(part 1 of 3)
# Autodesk Inventor assembly: CNC-FullAssembly
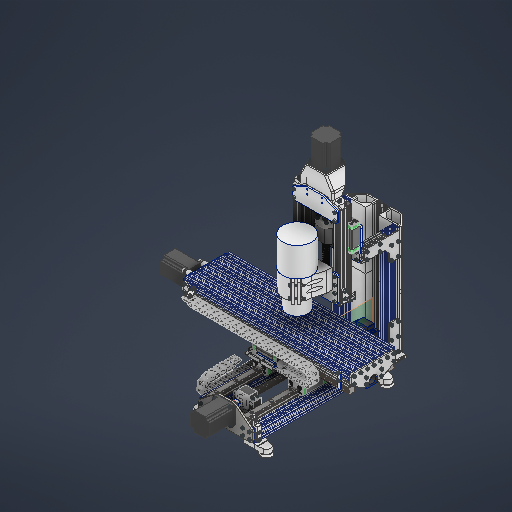
[picture p0: Inventor's stored thumbnail of the model, 512x512]
Saved by Autodesk Inventor 2026.2 (Build 302298000, 298)
## iProperties
Created: 2026-06-14
Part Number: CNC-FullAssembly
Document SubType Name: Assembly
Designer: Kenji
Mass: 17887.4 g
Surface Area: 25590.9 cm^2
Volume: 4676.24 cm^3
Author: Kenji
## Documents named in this file (79)
- C:\Users\Kenji\Documents\GitHub\DiyCNC-\CNC-FullAssembly.iam
- C:\Users\Kenji\Documents\GitHub\DiyCNC-\COTS-Parts\40x40x500mm-Extrusion.ipt
- C:\Users\Kenji\Documents\GitHub\DiyCNC-\COTS-Parts\SFU1605-BallScrewNut.iam
- C:\Users\Kenji\Documents\GitHub\DiyCNC-\COTS-Parts\DSG16H-BallScrewFixtureBlock.ipt
- C:\Users\Kenji\Documents\GitHub\DiyCNC-\COTS-Parts\SFU1605-BallScrew500mm.ipt
- C:\Users\Kenji\Documents\GitHub\DiyCNC-\COTS-Parts\BK12-BallScrewStabilizer.iam
- C:\Users\Kenji\Documents\GitHub\DiyCNC-\COTS-Parts\HGR20R-LinearRail500mm.ipt
- C:\Users\Kenji\Documents\GitHub\DiyCNC-\COTS-Parts\HGH20-LinearRailCarriage.iam
- C:\Users\Kenji\Documents\GitHub\DiyCNC-\COTS-Parts\91274A131_M5x20mm.ipt
- C:\Users\Kenji\Documents\GitHub\DiyCNC-\COTS-Parts\91290A231-M5x15mm.ipt
- C:\Users\Kenji\Documents\GitHub\DiyCNC-\COTS-Parts\Nema23-StepperMotor.ipt
- C:\Users\Kenji\Documents\GitHub\DiyCNC-\COTS-Parts\MH2025-6.35x10mmCoupler.iam
- C:\Users\Kenji\Documents\GitHub\DiyCNC-\COTS-Parts\BF12-BallScrewStabilizer2.ipt
- C:\Users\Kenji\Documents\GitHub\DiyCNC-\CNC-000-StructureGusset1.ipt
- C:\Users\Kenji\Documents\GitHub\DiyCNC-\COTS-Parts\20x40x500mm-Extrusion.ipt
- C:\Users\Kenji\Documents\GitHub\DiyCNC-\CNC-001-StructureGusset2.ipt
- C:\Users\Kenji\Documents\GitHub\DiyCNC-\CNC-002-ShimStructureGusset2.ipt
- C:\Users\Kenji\Documents\GitHub\DiyCNC-\COTS-Parts\90576A104-M5-NylockNut.ipt
- C:\Users\Kenji\Documents\GitHub\DiyCNC-\COTS-Parts\91292A195-M5x45mm.ipt
- C:\Users\Kenji\Documents\GitHub\DiyCNC-\CNC-003-StructureGusset3.ipt
- C:\Users\Kenji\Documents\GitHub\DiyCNC-\CNC-004-Nema23Shim.ipt
- C:\Users\Kenji\Documents\GitHub\DiyCNC-\COTS-Parts\91274A125-M5x8mm.ipt
- C:\Users\Kenji\Documents\GitHub\DiyCNC-\CNC-005-XAxisMount1.ipt
- C:\Users\Kenji\Documents\GitHub\DiyCNC-\COTS-Parts\91263A832-M5x10mm-Countersink.ipt
- C:\Users\Kenji\Documents\GitHub\DiyCNC-\CNC-006-XAxisMount2.ipt
- C:\Users\Kenji\Documents\GitHub\DiyCNC-\COTS-Parts\92095A495-M8-18mm-ButtonHead.ipt
- C:\Users\Kenji\Documents\GitHub\DiyCNC-\COTS-Parts\94645A210-M8-NylockNut.ipt
- C:\Users\Kenji\Documents\GitHub\DiyCNC-\COTS-Parts\20x40x500mm-Extrusion2.ipt
- C:\Users\Kenji\Documents\GitHub\DiyCNC-\COTS-Parts\20x20x500mm_Extrusion.ipt
- C:\Users\Kenji\Documents\GitHub\DiyCNC-\CNC-007-XAxisBallScrewMount.ipt
- C:\Users\Kenji\Documents\GitHub\DiyCNC-\CNC-008-XAxisNema23Mount.ipt
- C:\Users\Kenji\Documents\GitHub\DiyCNC-\CNC-009-XAxisNema23Spacer.ipt
- C:\Users\Kenji\Documents\GitHub\DiyCNC-\COTS-Parts\91290A198-M5-50mm.ipt
- C:\Users\Kenji\Documents\GitHub\DiyCNC-\COTS-Parts\3103-0001-0002-GobildaLimitSwitch.ipt
- C:\Users\Kenji\Documents\GitHub\DiyCNC-\CNC-010-XAxisLimitSwitchMount.ipt
- C:\Users\Kenji\Documents\GitHub\DiyCNC-\CNC-011-XAxisHardStop.ipt
- C:\Users\Kenji\Documents\GitHub\DiyCNC-\COTS-Parts\HGR20R-LinearRail300mm.ipt
- C:\Users\Kenji\Documents\GitHub\DiyCNC-\COTS-Parts\SFU1605-BallScrew400mm.ipt
- C:\Users\Kenji\Documents\GitHub\DiyCNC-\COTS-Parts\RouterSpindle-65mm.ipt
- C:\Users\Kenji\Documents\GitHub\DiyCNC-\COTS-Parts\90128A046-#2-.375in.ipt
- C:\Users\Kenji\Documents\GitHub\DiyCNC-\COTS-Parts\90480A003-#2-HexNut.ipt
- C:\Users\Kenji\Documents\GitHub\DiyCNC-\CNC-012-YAxisLimitSwitchMount.ipt
- C:\Users\Kenji\Documents\GitHub\DiyCNC-\COTS-Parts\20x40x100mm-Extrusion.ipt
- C:\Users\Kenji\Documents\GitHub\DiyCNC-\COTS-Parts\20x40x128mm-Extrusion.ipt
- C:\Users\Kenji\Documents\GitHub\DiyCNC-\CNC-013-ZAxisMainMount.ipt
- C:\Users\Kenji\Documents\GitHub\DiyCNC-\COTS-Parts\91274A134-M5x30mm.ipt
- C:\Users\Kenji\Documents\GitHub\DiyCNC-\COTS-Parts\92981A790-M5x40mm-ShoulderBolt.ipt
- C:\Users\Kenji\Documents\GitHub\DiyCNC-\COTS-Parts\HGR20R-LinearRail200mm.ipt
- C:\Users\Kenji\Documents\GitHub\DiyCNC-\COTS-Parts\SFU1605-BallScrew300mm.ipt
- C:\Users\Kenji\Documents\GitHub\DiyCNC-\CNC-014-ZAxisSubMount1.ipt
- C:\Users\Kenji\Documents\GitHub\DiyCNC-\COTS-Parts\90327A125-M5x10mm-LowProfileSCS.ipt
- C:\Users\Kenji\Documents\GitHub\DiyCNC-\COTS-Parts\91290A195-M5x35mm.ipt
- C:\Users\Kenji\Documents\GitHub\DiyCNC-\CNC-015-65mmSpindleMount.ipt
- C:\Users\Kenji\Documents\GitHub\DiyCNC-\COTS-Parts\20x20x250mm_Extrusion.ipt
- C:\Users\Kenji\Documents\GitHub\DiyCNC-\CNC-016-SpindleMountPlate.ipt
- C:\Users\Kenji\Documents\GitHub\DiyCNC-\CNC-017-SpindleMountPlate2.ipt
- C:\Users\Kenji\Documents\GitHub\DiyCNC-\CNC-018-ZAxisBallScrewStabilizerShim1.ipt
- C:\Users\Kenji\Documents\GitHub\DiyCNC-\CNC-019-ZAxisBallScrewStabilizerShim2.ipt
- C:\Users\Kenji\Documents\GitHub\DiyCNC-\CNC-020-ZAxisNema23Mount.ipt
- C:\Users\Kenji\Documents\GitHub\DiyCNC-\COTS-Parts\20x40x350mm-ExtrusionNoHoles.ipt
- C:\Users\Kenji\Documents\GitHub\DiyCNC-\CNC-021-ZAxisLimitSwitchMount.ipt
- C:\Users\Kenji\Documents\GitHub\DiyCNC-\CNC-022-XAxisBallScrewStabilizerMount.ipt
- C:\Users\Kenji\Documents\GitHub\DiyCNC-\CNC-023-YAxisBallScrewStabilizerMount.ipt
- C:\Users\Kenji\Documents\GitHub\DiyCNC-\CNC-024-MillFeet.ipt
- C:\Users\Kenji\Documents\GitHub\DiyCNC-\COTS-Parts\10x15-CableCarrierYAxis-2924-1015-1000.iam
- C:\Users\Kenji\Documents\GitHub\DiyCNC-\CNC-025-YAxisCableCarrierMount.ipt
- C:\Users\Kenji\Documents\GitHub\DiyCNC-\COTS-Parts\91274A117-M4x10mm.ipt
- C:\Users\Kenji\Documents\GitHub\DiyCNC-\CNC-026-CableCarrierTrack.ipt
- C:\Users\Kenji\Documents\GitHub\DiyCNC-\CNC-027-XAxisWireDuct.ipt
- C:\Users\Kenji\Documents\GitHub\DiyCNC-\CNC-028-WireTrack1.ipt
- C:\Users\Kenji\Documents\GitHub\DiyCNC-\CNC-028-WireTrack1_MIR.ipt
- C:\Users\Kenji\Documents\GitHub\DiyCNC-\COTS-Parts\10x15-CarbleCarrierXAxis-2924-1015-1000.iam
- C:\Users\Kenji\Documents\GitHub\DiyCNC-\COTS-Parts\94500A264-M3-12mm-ButtonHead.ipt
- C:\Users\Kenji\Documents\GitHub\DiyCNC-\COTS-Parts\90576A102-M3-NylockNut.ipt
- C:\Users\Kenji\Documents\GitHub\DiyCNC-\CNC-030-XAxisCableCarrierMount.ipt
- C:\Users\Kenji\Documents\GitHub\DiyCNC-\CNC-031-BackCover1.ipt
- C:\Users\Kenji\Documents\GitHub\DiyCNC-\CNC-031-BackCover1_MIR.ipt
- C:\Users\Kenji\Documents\GitHub\DiyCNC-\CNC-031-BackCover1_MIR2.ipt
- C:\Users\Kenji\Documents\GitHub\DiyCNC-\CNC-031-BackCover1_MIR_MIR3.ipt
## Components (468 placed, 78 different names)
1. 40x40x500mm-Extrusion:1 — Mate:1, Mate:2, Flush:1, Flush:2, Flush:3, Angle:1, Angle:3, Angle:4, Flush:20, Flush:21, Mate:48, Mate:49, Flush:35, Mate:264, Mate:286, Flush:146, Mate:293, Tangent:7, Tangent:13, Tangent:14, Flush:289, Mate:592, Mate:593, Flush:291, Mate:624, Flush:316, Tangent:17
2. 40x40x500mm-Extrusion:2 — Flush:2, Flush:3, Angle:2, Mate:39, Mate:40, Mate:41, Flush:22, Flush:23, Flush:38, Mate:290, Flush:147, Mate:294, Mate:299, Angle:26, Tangent:15, Mate:594, Flush:292, Angle:27, Angle:28, Mate:600, Flush:299, Angle:29, Mate:608, Tangent:16
3. SFU1605-BallScrewNut:1 [sub-assembly] — Mate:3, Mate:4, Mate:5, Mate:21, Mate:22, Mate:23, Mate:24, Mate:25, Mate:26, Mate:27
4. DSG16H-BallScrewFixtureBlock:1 — Mate:3, Mate:4, Mate:5, Angle:1, Flush:14, Mate:20, Angle:6, Mate:98, Mate:99
5. BK12-BallScrewStabilizer:1 [sub-assembly] — Angle:2, Mate:295, Mate:296, Mate:573, Mate:574, Mate:575, Mate:582, Mate:583, Mate:584, Mate:585, Mate:586
6. HGH20-LinearRailCarriage:1 [sub-assembly] — Flush:10, Flush:11, Mate:18, Flush:14, Mate:100, Mate:284, Mate:303, Mate:304
7. HGH20-LinearRailCarriage:2 [sub-assembly] — Flush:12, Flush:13, Mate:283, Mate:329
8. HGH20-LinearRailCarriage:3 [sub-assembly] — Flush:10, Flush:12, Mate:20, Mate:281, Mate:282
9. HGH20-LinearRailCarriage:4 [sub-assembly] — Flush:11, Mate:18, Flush:13, Mate:285
10. 91274A131_M5x20mm:1 — Mate:21, Mate:22, Flush:17, Flush:18
11. 91274A131_M5x20mm:2 — Mate:26, Flush:15, Flush:16
12. 91274A131_M5x20mm:3 — Mate:27, Flush:15
13. 91274A131_M5x20mm:4 — Mate:25, Flush:16, Flush:17
14. 91274A131_M5x20mm:5 — Mate:23, Flush:18, Flush:19
15. 91274A131_M5x20mm:6 — Mate:24, Flush:19
16. Nema23-StepperMotor:1 — Mate:32, Angle:3, Mate:33, Mate:59, Mate:60, Mate:61, Mate:62, Mate:63, Mate:301
17. MH2025-6.35x10mmCoupler:1 [sub-assembly] — Mate:32, Mate:33, Mate:297
18. BF12-BallScrewStabilizer2:1 — Angle:4, Mate:56, Mate:57, Mate:58, Mate:269, Mate:298, Mate:443, Mate:444, Mate:445, Mate:446, Mate:447
19. CNC-000-StructureGusset1:1 — Mate:39, Mate:40, Mate:41, Mate:42, Mate:43, Mate:44, Mate:45, Mate:65, Mate:77, Mate:79, Mate:265, Mate:287, Mate:291, Mate:302
20. 20x40x500mm-Extrusion:1 — Flush:20, Flush:21, Mate:75, Flush:36, Mate:293, Tangent:8, Flush:156, Flush:157, Mate:331, Mate:520, Mate:669, Mate:672, Mate:678, Mate:685, Mate:686, Mate:687
21. 20x40x500mm-Extrusion:2 — Flush:22, Flush:23, Mate:76, Flush:37, Mate:294, Mate:329, Mate:330, Flush:154, Flush:155, Mate:352, Tangent:9, Flush:255, Mate:679, Mate:680, Mate:681
22. CNC-001-StructureGusset2:1 — Mate:48, Mate:49, Mate:51, Mate:52, Mate:53, Mate:54, Mate:55, Mate:269, Mate:299, Mate:300, Mate:452
23. 91290A231-M5x15mm:27 — Mate:51, Mate:52, Flush:25, Flush:26
24. 91290A231-M5x15mm:28 — Mate:54, Flush:24, Flush:25
25. 91290A231-M5x15mm:29 — Mate:55, Flush:24
26. 91290A231-M5x15mm:30 — Mate:53, Flush:26
27. CNC-002-ShimStructureGusset2:1 — Mate:56, Mate:57, Mate:58, Mate:300
28. 91274A131_M5x20mm:7 — Mate:60, Flush:29, Mate:67
29. 91274A131_M5x20mm:8 — Mate:62, Mate:63, Flush:27, Mate:68
30. 91274A131_M5x20mm:9 — Mate:59, Flush:28, Flush:29, Mate:64
31. 91274A131_M5x20mm:10 — Mate:61, Flush:27, Flush:28, Mate:66
32. 90576A104-M5-NylockNut:1 — Mate:64, Mate:65, Flush:32
33. 90576A104-M5-NylockNut:2 — Mate:66, Flush:30, Mate:78, Mate:265
34. 90576A104-M5-NylockNut:3 — Mate:68, Flush:30, Flush:31
35. 90576A104-M5-NylockNut:4 — Mate:67, Flush:31, Flush:32
36. CNC-003-StructureGusset3:1 — Mate:75, Flush:35, Flush:36, Mate:80, Mate:81, Mate:82, Mate:83, Symmetry:1, Mate:640, Mate:641, Mate:642
37. CNC-003-StructureGusset3:2 — Mate:76, Flush:37, Flush:38, Mate:84, Mate:85, Mate:86, Mate:87, Flush:314, Flush:315, Symmetry:1
38. CNC-004-Nema23Shim:1 — Mate:77, Mate:78, Mate:79, Mate:301
39. HGH20-LinearRailCarriage:5 [sub-assembly] — Mate:91, Mate:92, Mate:131, Mate:132, Mate:133, Flush:142
40. HGH20-LinearRailCarriage:6 [sub-assembly] — Mate:128, Mate:129, Mate:130
41. HGH20-LinearRailCarriage:7 [sub-assembly] — Mate:125, Mate:126, Mate:127
42. HGH20-LinearRailCarriage:8 [sub-assembly] — Mate:134, Mate:135, Mate:136, Mate:137, Mate:138
43. HGR20R-LinearRail500mm:3 — Flush:50, Mate:137, Mate:138, Mate:202, Mate:226, Mate:314
44. HGR20R-LinearRail500mm:4 — Mate:91, Mate:92, Flush:50, Flush:106, Flush:107, Mate:199, Flush:119, Angle:10, Mate:224, Mate:225, Flush:142, Mate:313
45. DSG16H-BallScrewFixtureBlock:2 — Angle:6, Mate:94, Mate:95, Mate:96, Mate:97, Mate:121, Mate:122, Mate:123
46. SFU1605-BallScrewNut:2 [sub-assembly] — Mate:94, Mate:95, Mate:96, Mate:139, Mate:140, Mate:141, Mate:142, Mate:143, Mate:144, Mate:145
47. SFU1605-BallScrew500mm:2 — Mate:97, Mate:203, Mate:204, Mate:205, Mate:207, Mate:209, Mate:256
48. CNC-005-XAxisMount1:1 — Mate:98, Mate:99, Mate:100, Mate:101, Flush:53, Mate:102, Mate:103, Mate:104, Mate:105, Mate:106, Mate:107, Mate:108, Flush:57, Flush:58, Flush:59, Flush:60, Mate:109, Mate:110, Mate:111, Mate:112, Flush:61, Flush:63, Mate:113, Mate:114, Mate:115, Mate:116, Flush:65, Flush:66, Flush:67, Flush:68, Mate:117, Mate:118, Mate:119, Mate:120, Flush:69, Flush:70, Flush:71, Flush:72, Mate:124, Angle:7, Mate:166, Mate:177, Mate:179, Mate:181, Mate:183, Mate:186, Mate:187, Mate:190, Mate:191, Mate:282, Mate:283, Mate:285
49. 91263A832-M5x10mm-Countersink:1 — Mate:101, Flush:53, Flush:56
50. 91263A832-M5x10mm-Countersink:2 — Mate:104, Flush:55, Mate:281
51. 91263A832-M5x10mm-Countersink:3 — Mate:102, Flush:54, Flush:55, Flush:56
52. 91263A832-M5x10mm-Countersink:4 — Mate:103, Flush:54
53. 91263A832-M5x10mm-Countersink:5 — Mate:105, Flush:59
54. 91263A832-M5x10mm-Countersink:6 — Mate:106, Flush:58, Mate:284
55. 91263A832-M5x10mm-Countersink:7 — Mate:108, Flush:57
56. 91263A832-M5x10mm-Countersink:8 — Mate:107, Flush:60
57. 91263A832-M5x10mm-Countersink:9 — Mate:112, Flush:62
58. 91263A832-M5x10mm-Countersink:10 — Mate:111, Flush:61, Flush:62
59. 91263A832-M5x10mm-Countersink:11 — Mate:109, Flush:63, Flush:64
60. 91263A832-M5x10mm-Countersink:12 — Mate:110, Flush:64
61. 91263A832-M5x10mm-Countersink:13 — Mate:113, Flush:65
62. 91263A832-M5x10mm-Countersink:14 — Mate:116, Flush:67
63. 91263A832-M5x10mm-Countersink:15 — Mate:115, Flush:66
64. 91263A832-M5x10mm-Countersink:16 — Mate:114, Flush:68
65. 91263A832-M5x10mm-Countersink:17 — Mate:118, Flush:71
66. 91263A832-M5x10mm-Countersink:18 — Mate:119, Flush:69
67. 91263A832-M5x10mm-Countersink:19 — Mate:117, Flush:72
68. 91263A832-M5x10mm-Countersink:20 — Mate:120, Flush:70
69. CNC-006-XAxisMount2:1 — Mate:121, Mate:122, Mate:123, Mate:124, Angle:7, Mate:125, Mate:126, Mate:127, Mate:128, Mate:129, Mate:130, Mate:131, Mate:132, Mate:133, Mate:134, Mate:135, Mate:136, Mate:146, Mate:147, Mate:148, Mate:149, Flush:78, Flush:79, Flush:81, Mate:150, Mate:151, Mate:152, Mate:153, Flush:82, Flush:83, Flush:84, Flush:85, Mate:154, Mate:155, Mate:156, Mate:157, Flush:86, Flush:87, Mate:158, Mate:159, Mate:160, Mate:161, Flush:90, Flush:91, Flush:92, Flush:93, Mate:162, Mate:163, Mate:164, Mate:165, Flush:94, Flush:95, Flush:96, Flush:97, Mate:166, Mate:167, Mate:168, Mate:169, Mate:170, Mate:171, Mate:172, Mate:173, Mate:174, Mate:175, Mate:602, Mate:603, Mate:604, Mate:616, Mate:618, Mate:619, Angle:30, Mate:644, Mate:645, Mate:653
70. 91274A131_M5x20mm:11 — Mate:139, Mate:140, Flush:74, Flush:75
71. 91274A131_M5x20mm:12 — Mate:145, Flush:76, Flush:77
72. 91274A131_M5x20mm:13 — Mate:144, Flush:77
73. 91274A131_M5x20mm:14 — Mate:141, Flush:73, Flush:74
74. 91274A131_M5x20mm:15 — Mate:143, Flush:75
75. 91274A131_M5x20mm:16 — Mate:142, Flush:73, Flush:76
76. 91263A832-M5x10mm-Countersink:21 — Mate:149, Flush:78
77. 91263A832-M5x10mm-Countersink:22 — Mate:146, Flush:80
78. 91263A832-M5x10mm-Countersink:23 — Mate:147, Flush:79, Flush:80
79. 91263A832-M5x10mm-Countersink:24 — Mate:148, Flush:81
80. 91263A832-M5x10mm-Countersink:25 — Mate:150, Flush:85
81. 91263A832-M5x10mm-Countersink:26 — Mate:153, Flush:83
82. 91263A832-M5x10mm-Countersink:27 — Mate:151, Flush:82
83. 91263A832-M5x10mm-Countersink:28 — Mate:152, Flush:84
84. 91263A832-M5x10mm-Countersink:29 — Mate:156, Flush:87, Flush:88
85. 91263A832-M5x10mm-Countersink:30 — Mate:155, Flush:89
86. 91263A832-M5x10mm-Countersink:31 — Mate:154, Flush:88, Flush:89
87. 91263A832-M5x10mm-Countersink:32 — Mate:157, Flush:86
88. 91263A832-M5x10mm-Countersink:33 — Mate:159, Flush:93
89. 91263A832-M5x10mm-Countersink:34 — Mate:160, Flush:91
90. 91263A832-M5x10mm-Countersink:35 — Mate:158, Flush:92
91. 91263A832-M5x10mm-Countersink:36 — Mate:161, Flush:90
92. 91263A832-M5x10mm-Countersink:37 — Mate:164, Flush:95
93. 91263A832-M5x10mm-Countersink:38 — Mate:162, Flush:96
94. 91263A832-M5x10mm-Countersink:39 — Mate:163, Flush:97
95. 91263A832-M5x10mm-Countersink:40 — Mate:165, Flush:94
96. 92095A495-M8-18mm-ButtonHead:1 — Mate:167, Flush:98, Flush:99, Flush:102, Mate:176
97. 92095A495-M8-18mm-ButtonHead:2 — Mate:168, Flush:99, Flush:104, Mate:178
98. 92095A495-M8-18mm-ButtonHead:3 — Mate:169, Mate:170, Flush:98, Flush:100, Mate:180
99. 92095A495-M8-18mm-ButtonHead:8 — Mate:171, Flush:100, Mate:182
100. 92095A495-M8-18mm-ButtonHead:9 — Mate:174, Flush:103, Flush:104, Mate:188
101. 92095A495-M8-18mm-ButtonHead:10 — Mate:175, Flush:103, Mate:189
102. 92095A495-M8-18mm-ButtonHead:11 — Mate:172, Flush:101, Flush:102, Mate:184
103. 92095A495-M8-18mm-ButtonHead:12 — Mate:173, Flush:101, Mate:185
104. 94645A210-M8-NylockNut:1 — Mate:176, Mate:177
105. 94645A210-M8-NylockNut:2 — Mate:178, Mate:179
106. 94645A210-M8-NylockNut:3 — Mate:180, Mate:181
107. 94645A210-M8-NylockNut:4 — Mate:182, Mate:183
108. 94645A210-M8-NylockNut:5 — Mate:184, Mate:187
109. 94645A210-M8-NylockNut:6 — Mate:185, Mate:186
110. 94645A210-M8-NylockNut:7 — Mate:188, Mate:191
111. 94645A210-M8-NylockNut:8 — Mate:189, Mate:190
112. 20x40x500mm-Extrusion2:1 — Flush:106, Flush:107, Flush:108, Mate:193, Flush:109, Flush:116, Flush:117, Mate:200, Mate:211, Mate:212, Mate:213, Angle:11, Tangent:2, Flush:143, Tangent:4, Mate:270, Mate:658, Mate:668
113. 20x40x500mm-Extrusion2:2 — Flush:108, Mate:193, Flush:109, Flush:110, Flush:111, Mate:194, Angle:8, Angle:9, Mate:408, Mate:601
114. 20x40x500mm-Extrusion2:3 — Flush:110, Flush:111, Mate:194, Mate:201, Flush:118, Mate:228, Mate:229
115. 20x20x500mm_Extrusion:3 — Flush:116, Mate:199, Flush:117, Mate:200, Tangent:3, Tangent:5, Flush:144, Mate:312, Angle:32
116. 20x40x500mm-Extrusion2:4 — Mate:201, Flush:118, Mate:202, Mate:227, Mate:276
117. BF12-BallScrewStabilizer2:2 — Mate:203, Mate:204, Flush:119, Angle:8, Mate:543
118. Nema23-StepperMotor:2 — Mate:205, Angle:9, Mate:206, Mate:208, Mate:243, Mate:244, Mate:245, Mate:246, Mate:247
119. MH2025-6.35x10mmCoupler:2 [sub-assembly] — Mate:206, Mate:207, Mate:208, Mate:240
120. BK12-BallScrewStabilizer:2 [sub-assembly] — Mate:209, Angle:10, Mate:256, Mate:557, Mate:558, Mate:559, Mate:570
121. CNC-007-XAxisBallScrewMount:1 — Mate:211, Mate:212, Mate:213, Mate:214, Mate:215, Mate:216, Mate:217, Mate:218, Mate:219, Mate:220, Mate:221, Mate:222, Mate:223, Mate:529, Mate:530, Mate:531, Mate:532, Mate:533
122. 91290A231-M5x15mm:31 — Mate:219, Flush:123, Flush:124
123. 91290A231-M5x15mm:32 — Mate:218, Flush:122, Flush:123, Flush:125, Flush:127
124. 91290A231-M5x15mm:33 — Mate:215, Flush:120, Flush:121
125. 91290A231-M5x15mm:34 — Mate:216, Flush:120
126. 91290A231-M5x15mm:35 — Mate:220, Flush:124
127. 91290A231-M5x15mm:36 — Mate:214, Mate:221, Flush:125, Flush:126
128. 91290A231-M5x15mm:37 — Mate:217, Flush:121, Flush:122
129. 91290A231-M5x15mm:38 — Mate:222, Flush:126
130. 91290A231-M5x15mm:39 — Mate:223, Flush:127
131. CNC-008-XAxisNema23Mount:1 — Mate:227, Mate:228, Mate:229, Mate:230, Mate:231, Mate:232, Mate:233, Mate:234, Mate:235, Mate:236, Mate:237, Mate:238, Mate:239, Mate:241, Mate:242, Mate:252, Mate:253, Mate:254, Mate:255
132. 91290A231-M5x15mm:58 — Mate:233, Flush:133, Flush:134
133. 91290A231-M5x15mm:59 — Mate:231, Flush:134, Flush:135
134. 91290A231-M5x15mm:60 — Mate:232, Flush:136
135. 91290A231-M5x15mm:61 — Mate:234, Flush:132, Flush:133
136. 91290A231-M5x15mm:62 — Mate:235, Flush:131, Flush:132
137. 91290A231-M5x15mm:63 — Mate:238, Mate:239, Flush:129
138. 91290A231-M5x15mm:64 — Mate:230, Flush:135, Flush:136
139. 91290A231-M5x15mm:65 — Mate:237, Flush:129, Flush:130
140. 91290A231-M5x15mm:66 — Mate:236, Flush:130, Flush:131
141. CNC-009-XAxisNema23Spacer:1 — Mate:240, Mate:241, Mate:242
142. 91290A198-M5-50mm:1 — Mate:244, Flush:138, Mate:248
143. 91290A198-M5-50mm:2 — Mate:243, Flush:138, Flush:139, Mate:250
144. 91290A198-M5-50mm:3 — Mate:245, Flush:137, Flush:139, Mate:251
145. 91290A198-M5-50mm:4 — Mate:246, Mate:247, Flush:137, Mate:249
146. 90576A104-M5-NylockNut:5 — Mate:251, Mate:252
147. 90576A104-M5-NylockNut:6 — Mate:248, Mate:254
148. 90576A104-M5-NylockNut:7 — Mate:250, Mate:255
149. 90576A104-M5-NylockNut:8 — Mate:249, Mate:253
150. 3103-0001-0002-GobildaLimitSwitch:1 — Angle:11, Mate:258, Mate:259, Mate:305, Mate:306, Mate:310
151. CNC-010-XAxisLimitSwitchMount:1 — Tangent:2, Mate:258, Mate:259, Tangent:3, Flush:143, Mate:307, Mate:308, Mate:312, Mate:415, Mate:416, Mate:420
152. CNC-011-XAxisHardStop:1 — Tangent:4, Tangent:5, Mate:270, Flush:144, Mate:271, Mate:272, Mate:273, Mate:274
153. 91274A125-M5x8mm:25 — Mate:271, Mate:272, Flush:145
154. 91274A125-M5x8mm:26 — Mate:273, Flush:145, Mate:275
155. CNC-011-XAxisHardStop:2 — Mate:274, Mate:275, Mate:276, Mate:277, Mate:278, Mate:279, Mate:280
156. 91274A125-M5x8mm:27 — Mate:277, Mate:280
157. 91274A125-M5x8mm:28 — Mate:278, Mate:279
158. HGR20R-LinearRail300mm:1 — Mate:290, Mate:291, Flush:147, Mate:292
159. HGR20R-LinearRail300mm:2 — Mate:286, Flush:146, Mate:287, Mate:288, Mate:289, Mate:303, Mate:304
160. SFU1605-BallScrew400mm:1 — Mate:295, Mate:296, Mate:297, Mate:298
161. RouterSpindle-65mm:1 — Tangent:7, Tangent:8, Flush:191, Mate:408, Mate:453, Mate:454
162. 90128A046-#2-.375in:1 — Mate:305, Mate:308, Mate:311
163. 90128A046-#2-.375in:2 — Mate:306, Mate:307, Mate:309
164. 90480A003-#2-HexNut:1 — Mate:309, Mate:310, Flush:149
165. 90480A003-#2-HexNut:2 — Mate:311, Flush:149
166. 20x40x100mm-Extrusion:3 — Mate:330, Flush:154, Flush:155, Mate:336, Flush:160, Flush:161, Tangent:10, Angle:17, Flush:185, Mate:387
167. 20x40x100mm-Extrusion:4 — Flush:156, Flush:157, Mate:331, Mate:355, Flush:186
168. 20x40x128mm-Extrusion:1 — Mate:336, Flush:160, Flush:161, Mate:349, Angle:19, Mate:378
169. 91274A125-M5x8mm:29 — Flush:165, Mate:356, Flush:170, Flush:171, Flush:172
170. 91274A125-M5x8mm:30 — Flush:165, Mate:357, Mate:358
171. 91274A125-M5x8mm:31 — Mate:363, Flush:173, Flush:175, Flush:176
172. 91274A125-M5x8mm:32 — Mate:364, Mate:365, Flush:173, Flush:325
173. HGH20-LinearRailCarriage:9 [sub-assembly] — Mate:349, Flush:180, Flush:181, Angle:18, Flush:185, Mate:383, Mate:384, Mate:387
174. HGH20-LinearRailCarriage:10 [sub-assembly] — Flush:180, Flush:181, Flush:186, Mate:385, Mate:386, Flush:198, Mate:409, Mate:410, Mate:411, Mate:412
175. CNC-013-ZAxisMainMount:1 — Mate:353, Mate:354, Mate:355, Mate:356, Mate:357, Mate:358, Mate:359, Mate:360, Mate:361, Mate:362, Mate:370, Mate:371, Mate:372
176. CNC-013-ZAxisMainMount:2 — Mate:352, Tangent:9, Tangent:10, Angle:17, Mate:353, Mate:354, Mate:363, Mate:364, Mate:365, Mate:366, Mate:367, Mate:368, Mate:369, Mate:373, Mate:374, Mate:375
177. 91274A125-M5x8mm:33 — Mate:359, Flush:172
178. 91274A125-M5x8mm:34 — Mate:360, Flush:171
179. 91274A125-M5x8mm:35 — Mate:362, Flush:169
180. 91274A125-M5x8mm:36 — Mate:361, Flush:169, Flush:170
181. 91274A125-M5x8mm:37 — Mate:366, Flush:176
182. 91274A125-M5x8mm:38 — Mate:369, Flush:174, Flush:175
183. 91274A125-M5x8mm:39 — Mate:368, Flush:174
184. 91274A125-M5x8mm:40 — Mate:367, Flush:325
185. 91274A134-M5x30mm:1 — Mate:373, Flush:178
186. 91274A134-M5x30mm:2 — Mate:374, Mate:375, Flush:178
187. 91274A134-M5x30mm:3 — Mate:370, Flush:177
188. 91274A134-M5x30mm:4 — Mate:371, Mate:372, Flush:177
189. DSG16H-BallScrewFixtureBlock:3 — Angle:18, Mate:376, Angle:19, Mate:378, Mate:388, Mate:389, Mate:390, Flush:198, Mate:409
190. BF12-BallScrewStabilizer2:3 — Mate:376, Mate:379, Mate:380, Mate:381, Mate:382, Flush:199, Angle:20, Mate:399, Angle:21, Mate:404, Mate:405, Mate:468, Mate:469, Mate:513, Mate:514
191. 92981A790-M5x40mm-ShoulderBolt:1 — Mate:380, Mate:381
192. 92981A790-M5x40mm-ShoulderBolt:2 — Mate:379, Mate:382
193. HGR20R-LinearRail200mm:1 — Mate:383, Mate:384, Flush:189, Flush:191, Mate:456, Flush:224, Mate:459, Mate:460, Mate:461, Mate:464
194. HGR20R-LinearRail200mm:2 — Mate:385, Mate:386, Flush:189, Flush:199, Angle:20, Mate:455, Flush:222, Flush:223, Mate:457, Mate:458, Mate:462, Mate:463, Mate:465
195. SFU1605-BallScrewNut:3 [sub-assembly] — Mate:388, Mate:389, Mate:390, Mate:391, Mate:392, Mate:393, Mate:394, Mate:395, Mate:396, Mate:397
196. 91274A131_M5x20mm:17 — Mate:392, Flush:193
197. 91274A131_M5x20mm:18 — Mate:391, Mate:397, Flush:197
198. 91274A131_M5x20mm:19 — Mate:393, Flush:193, Flush:194
199. 91274A131_M5x20mm:20 — Mate:395, Flush:195, Flush:196
200. 91274A131_M5x20mm:21 — Mate:396, Flush:196
201. 91274A131_M5x20mm:22 — Mate:394, Flush:194, Flush:195, Flush:197
202. BK12-BallScrewStabilizer:3 [sub-assembly] — Mate:399, Angle:21, Mate:401, Angle:22, Mate:406, Mate:490, Mate:491, Mate:492, Mate:493, Mate:494, Mate:495, Mate:496, Mate:510, Mate:511
203. Nema23-StepperMotor:3 — Mate:402, Angle:22, Mate:403, Mate:524, Mate:525, Mate:526, Mate:527, Mate:528
204. MH2025-6.35x10mmCoupler:3 [sub-assembly] — Mate:401, Mate:402, Mate:403, Mate:407
205. SFU1605-BallScrew300mm:1 — Mate:404, Mate:405, Mate:406, Mate:407
206. CNC-014-ZAxisSubMount1:1 — Mate:410, Mate:411, Mate:412, Mate:421, Mate:422, Mate:423, Mate:424, Mate:425, Mate:426, Mate:427, Mate:428, Mate:429, Mate:430, Mate:431, Mate:432, Mate:433, Mate:434, Mate:435, Mate:436, Mate:437, Mate:438, Mate:439, Mate:440, Mate:441, Mate:442, Mate:466, Mate:467
207. 90327A125-M5x10mm-LowProfileSCS:1 — Mate:416, Flush:201
208. 90327A125-M5x10mm-LowProfileSCS:2 — Mate:415, Flush:201, Mate:420
209. 90327A125-M5x10mm-LowProfileSCS:5 — Mate:424, Mate:425, Flush:202
210. 90327A125-M5x10mm-LowProfileSCS:6 — Mate:423, Flush:204
211. 90327A125-M5x10mm-LowProfileSCS:7 — Mate:422, Flush:202, Flush:203
212. 90327A125-M5x10mm-LowProfileSCS:8 — Mate:421, Flush:203, Flush:204
213. 90327A125-M5x10mm-LowProfileSCS:9 — Mate:426, Flush:206, Flush:207
214. 90327A125-M5x10mm-LowProfileSCS:10 — Mate:429, Mate:430, Flush:205
215. 90327A125-M5x10mm-LowProfileSCS:11 — Mate:427, Flush:205, Flush:206
216. 90327A125-M5x10mm-LowProfileSCS:12 — Mate:428, Flush:207
217. 91290A231-M5x15mm:96 — Mate:431, Mate:432, Flush:210
218. 91290A231-M5x15mm:97 — Mate:435, Flush:208, Flush:209
219. 91290A231-M5x15mm:98 — Mate:434, Flush:209, Flush:210
220. 91290A231-M5x15mm:99 — Mate:433, Flush:208
221. 90327A125-M5x10mm-LowProfileSCS:13 — Mate:436, Mate:437, Flush:211, Flush:213, Flush:215
222. 90327A125-M5x10mm-LowProfileSCS:14 — Mate:438, Flush:211
223. 90327A125-M5x10mm-LowProfileSCS:15 — Mate:439, Flush:212, Flush:213
224. 90327A125-M5x10mm-LowProfileSCS:16 — Mate:440, Flush:212, Flush:234
225. 90327A125-M5x10mm-LowProfileSCS:17 — Mate:441, Flush:214, Flush:215
226. 90327A125-M5x10mm-LowProfileSCS:18 — Mate:442, Flush:214
227. 91290A195-M5x35mm:1 — Mate:445, Flush:218, Mate:451
228. 91290A195-M5x35mm:2 — Mate:443, Flush:216, Flush:217, Mate:448
229. 91290A195-M5x35mm:3 — Mate:446, Mate:447, Flush:216, Mate:449
230. 91290A195-M5x35mm:4 — Mate:444, Flush:217, Flush:218, Mate:450
231. 90576A104-M5-NylockNut:9 — Mate:448, Mate:452, Flush:219
232. 90576A104-M5-NylockNut:10 — Mate:449, Flush:219, Flush:220
233. 90576A104-M5-NylockNut:11 — Mate:450, Flush:221
234. 90576A104-M5-NylockNut:12 — Mate:451, Flush:220, Flush:221
235. CNC-015-65mmSpindleMount:1 — Mate:453, Mate:454, Angle:23, Mate:476, Mate:477, Mate:478, Mate:479, Mate:480, Mate:503, Mate:504, Mate:505, Mate:506, Mate:509
236. 20x20x250mm_Extrusion:1 — Mate:455, Flush:222, Flush:223, Flush:225, Angle:23, Mate:497, Mate:516, Mate:518, Angle:24, Angle:25, Tangent:12, Mate:556, Flush:273
237. 20x20x250mm_Extrusion:2 — Mate:456, Flush:224, Flush:225, Mate:470, Mate:517
238. 91290A231-M5x15mm:100 — Mate:457, Mate:458, Flush:227, Flush:228, Flush:231, Flush:232
239. 91290A231-M5x15mm:101 — Mate:459, Flush:228, Flush:229
240. 91290A231-M5x15mm:102 — Mate:460, Flush:229, Flush:230
241. 91290A231-M5x15mm:103 — Mate:461, Flush:230
242. 91290A231-M5x15mm:104 — Mate:462, Flush:226, Flush:227
243. 91290A231-M5x15mm:105 — Mate:463, Flush:226
244. 91290A231-M5x15mm:106 — Mate:464, Flush:232
245. 91290A231-M5x15mm:107 — Mate:465, Flush:231
246. 90327A125-M5x10mm-LowProfileSCS:19 — Mate:466, Flush:233, Flush:234
247. 90327A125-M5x10mm-LowProfileSCS:20 — Mate:467, Flush:233
248. CNC-016-SpindleMountPlate:1 — Mate:468, Mate:469, Mate:470, Mate:471, Mate:472, Mate:473, Mate:474, Mate:475, Mate:481, Mate:482, Mate:483, Mate:484, Mate:485, Mate:486, Mate:487, Mate:488, Mate:489, Mate:515
249. 90576A104-M5-NylockNut:13 — Mate:471, Mate:472, Flush:235, Flush:237
250. 90576A104-M5-NylockNut:14 — Mate:473, Flush:235
251. 90576A104-M5-NylockNut:15 — Mate:474, Flush:236, Flush:237
252. 90576A104-M5-NylockNut:16 — Mate:475, Flush:236
253. 91274A131_M5x20mm:23 — Mate:476, Flush:239, Flush:240, Mate:480
254. 91274A131_M5x20mm:24 — Mate:477, Flush:240
255. 91274A131_M5x20mm:25 — Mate:478, Flush:238
256. 91274A131_M5x20mm:26 — Mate:479, Flush:238, Flush:239
257. 90327A125-M5x10mm-LowProfileSCS:21 — Mate:481, Mate:482, Flush:241, Flush:247
258. 90327A125-M5x10mm-LowProfileSCS:22 — Mate:483, Flush:241, Flush:243
259. 90327A125-M5x10mm-LowProfileSCS:23 — Mate:484, Flush:242, Flush:243
260. 90327A125-M5x10mm-LowProfileSCS:24 — Mate:485, Flush:242
261. 90327A125-M5x10mm-LowProfileSCS:25 — Mate:488, Flush:244
262. 90327A125-M5x10mm-LowProfileSCS:26 — Mate:486, Flush:246, Flush:247
263. 90327A125-M5x10mm-LowProfileSCS:27 — Mate:487, Flush:245, Flush:246
264. 90327A125-M5x10mm-LowProfileSCS:28 — Mate:489, Flush:244, Flush:245
265. 92981A790-M5x40mm-ShoulderBolt:3 — Mate:491, Flush:250
266. 92981A790-M5x40mm-ShoulderBolt:4 — Mate:492, Flush:248, Flush:249
267. 92981A790-M5x40mm-ShoulderBolt:5 — Mate:490, Flush:249, Flush:250
268. 92981A790-M5x40mm-ShoulderBolt:6 — Mate:493, Mate:494, Flush:248
269. CNC-017-SpindleMountPlate2:1 — Mate:495, Mate:496, Mate:497, Mate:498, Mate:499, Mate:500, Mate:501, Mate:502, Mate:512
270. 90327A125-M5x10mm-LowProfileSCS:29 — Mate:499, Flush:252, Flush:253
271. 90327A125-M5x10mm-LowProfileSCS:30 — Mate:498, Flush:253
272. 90327A125-M5x10mm-LowProfileSCS:31 — Mate:500, Flush:251
273. 90327A125-M5x10mm-LowProfileSCS:32 — Mate:501, Mate:502, Flush:251, Flush:252
274. 91274A134-M5x30mm:5 — Mate:503, Mate:506, Mate:507
275. 91274A134-M5x30mm:6 — Mate:504, Mate:505, Mate:508
276. 90576A104-M5-NylockNut:17 — Mate:508, Mate:509, Flush:254
277. 90576A104-M5-NylockNut:18 — Mate:507, Flush:254
278. CNC-018-ZAxisBallScrewStabilizerShim1:1 — Mate:510, Mate:511, Mate:512
279. CNC-019-ZAxisBallScrewStabilizerShim2:1 — Mate:513, Mate:514, Mate:515
280. CNC-020-ZAxisNema23Mount:1 — Mate:516, Mate:517, Mate:518, Mate:521, Mate:522, Mate:523, Mate:538
281. 20x40x350mm-ExtrusionNoHoles:1 — Flush:255, Mate:520, Mate:669, Mate:671
282. 91274A131_M5x20mm:29 — Mate:521, Flush:256
283. 91274A131_M5x20mm:30 — Mate:522, Mate:523, Flush:256
284. 91274A131_M5x20mm:31 — Mate:525, Flush:257, Flush:258, Mate:534
285. 91274A131_M5x20mm:32 — Mate:524, Flush:259, Mate:535
286. 91274A131_M5x20mm:33 — Mate:526, Flush:258, Flush:259, Mate:537
287. 91274A131_M5x20mm:34 — Mate:527, Mate:528, Flush:257, Mate:536
288. 91274A134-M5x30mm:7 — Mate:532, Mate:533, Flush:260, Mate:539
289. 91274A134-M5x30mm:8 — Mate:531, Flush:262, Mate:542
290. 91274A134-M5x30mm:9 — Mate:530, Flush:260, Flush:261, Mate:540
291. 91274A134-M5x30mm:10 — Mate:529, Flush:261, Flush:262, Mate:541
292. 90576A104-M5-NylockNut:19 — Mate:535, Flush:263, Flush:264
293. 90576A104-M5-NylockNut:20 — Mate:534, Flush:264, Flush:265
294. 90576A104-M5-NylockNut:21 — Mate:537, Mate:538, Flush:263
295. 90576A104-M5-NylockNut:22 — Mate:536, Flush:265
296. 90576A104-M5-NylockNut:23 — Mate:542, Mate:543, Flush:266, Flush:267
297. 90576A104-M5-NylockNut:24 — Mate:539, Flush:267, Flush:268
298. 90576A104-M5-NylockNut:25 — Mate:541, Flush:266
299. 90576A104-M5-NylockNut:26 — Mate:540, Flush:268
300. 3103-0001-0002-GobildaLimitSwitch:3 — Angle:24, Angle:25, Mate:544, Mate:545, Mate:546, Mate:547, Mate:548, Mate:549
301. CNC-021-ZAxisLimitSwitchMount:1 — Mate:544, Mate:545, Tangent:12, Mate:546, Mate:552, Mate:553, Mate:554, Mate:555, Mate:556, Flush:273
302. 90480A003-#2-HexNut:5 — Mate:548, Flush:270, Mate:550
303. 90480A003-#2-HexNut:6 — Mate:547, Mate:549, Flush:270, Mate:551
304. 90128A046-#2-.375in:5 — Mate:550, Flush:271
305. 90128A046-#2-.375in:6 — Mate:551, Flush:271, Mate:552
306. 90327A125-M5x10mm-LowProfileSCS:33 — Mate:553, Flush:272
307. 90327A125-M5x10mm-LowProfileSCS:34 — Mate:554, Mate:555, Flush:272
308. CNC-022-XAxisBallScrewStabilizerMount:1 — Mate:557, Mate:558, Mate:559, Mate:560, Mate:561, Mate:562, Mate:563, Mate:564, Mate:565, Mate:566, Mate:567, Mate:601
309. 91290A195-M5x35mm:5 — Mate:560, Flush:274, Flush:275, Mate:571
310. 91290A195-M5x35mm:6 — Mate:561, Mate:562, Flush:274, Flush:276, Mate:568
311. 91290A195-M5x35mm:7 — Mate:564, Flush:276, Mate:569
312. 91290A195-M5x35mm:8 — Mate:563, Flush:275, Mate:572
313. 91274A125-M5x8mm:41 — Mate:565, Flush:277
314. 91274A125-M5x8mm:42 — Mate:566, Mate:567, Flush:277
315. 90576A104-M5-NylockNut:27 — Mate:568, Flush:278, Flush:279
316. 90576A104-M5-NylockNut:28 — Mate:569, Mate:570, Flush:278
317. 90576A104-M5-NylockNut:29 — Mate:571, Flush:279, Flush:280
318. 90576A104-M5-NylockNut:30 — Mate:572, Flush:280
319. CNC-023-YAxisBallScrewStabilizerMount:1 — Mate:573, Mate:574, Mate:575, Mate:576, Mate:577, Mate:578, Mate:579, Mate:580, Mate:581, Mate:588
320. 91290A231-M5x15mm:108 — Mate:576, Mate:577, Flush:281
321. 91290A231-M5x15mm:109 — Mate:579, Flush:282
322. 91290A231-M5x15mm:110 — Mate:578, Flush:281
323. 91290A231-M5x15mm:111 — Mate:580, Mate:581, Flush:282
324. 91292A195-M5x45mm:9 — Mate:586, Flush:285, Mate:589
325. 91292A195-M5x45mm:10 — Mate:582, Mate:583, Flush:283, Flush:284, Mate:590
326. 91292A195-M5x45mm:11 — Mate:585, Flush:284, Mate:591
327. 91292A195-M5x45mm:12 — Mate:584, Flush:283, Flush:285, Mate:587
328. 90576A104-M5-NylockNut:31 — Mate:587, Mate:588, Flush:286, Flush:287
329. 90576A104-M5-NylockNut:32 — Mate:591, Flush:288
330. 90576A104-M5-NylockNut:33 — Mate:589, Flush:286
331. 90576A104-M5-NylockNut:34 — Mate:590, Flush:287, Flush:288
332. CNC-024-MillFeet:1 — Tangent:13, Tangent:14, Flush:289, Mate:592, Flush:290, Mate:597
333. CNC-024-MillFeet:2 — Flush:290, Mate:593, Flush:291, Flush:295, Mate:598, Mate:599
334. CNC-024-MillFeet:3 — Angle:26, Tangent:15, Mate:594, Flush:292, Flush:293, Flush:294, Mate:596
335. CNC-024-MillFeet:4 — Flush:293, Flush:294, Flush:295, Mate:595
336. 10x15-CableCarrierYAxis-2924-1015-1000:1 [sub-assembly] — Angle:27, Angle:28, Mate:600, Flush:299, Mate:656
337. CNC-025-YAxisCableCarrierMount:1 — Mate:602, Mate:603, Mate:604, Mate:605, Mate:606, Mate:607, Mate:648, Mate:649, Mate:650, Mate:651
338. 91274A117-M4x10mm:1 — Mate:605, Mate:606, Flush:300
339. 91274A117-M4x10mm:2 — Mate:607, Flush:300
340. CNC-026-CableCarrierTrack:1 — Angle:29, Mate:608, Tangent:16, Flush:302, Flush:303, Flush:306, Mate:611, Mate:612
341. CNC-026-CableCarrierTrack:2 — Flush:302, Flush:303, Flush:305, Mate:613, Mate:614, Mate:615
342. CNC-026-CableCarrierTrack:3 — Flush:305, Flush:306, Mate:609, Mate:610
343. 91274A125-M5x8mm:43 — Mate:613, Flush:308, Flush:309
344. 91274A125-M5x8mm:44 — Mate:612, Flush:311, Flush:312
345. 91274A125-M5x8mm:45 — Mate:614, Mate:615, Flush:308
346. 91274A125-M5x8mm:46 — Mate:609, Flush:309, Flush:310, Flush:311
347. 91274A125-M5x8mm:47 — Mate:611, Flush:312
348. 91274A125-M5x8mm:48 — Mate:610, Flush:310
349. CNC-027-XAxisWireDuct:1 — Mate:616, Mate:618, Mate:620, Mate:621, Angle:30
350. 91274A117-M4x10mm:3 — Mate:619, Mate:620, Flush:313
351. 91274A117-M4x10mm:4 — Mate:621, Flush:313
352. CNC-028-WireTrack1:1 — Flush:314, Flush:315, Mate:622, Mate:623
353. CNC-012-YAxisLimitSwitchMount:2 — Mate:624, Flush:316, Tangent:17, Mate:625, Mate:626, Mate:627, Mate:628, Mate:629, Mate:633, Angle:31, Mate:636
354. 3103-0001-0002-GobildaLimitSwitch:4 — Mate:625, Mate:626, Mate:630, Mate:631, Mate:632, Mate:633
355. 90327A125-M5x10mm-LowProfileSCS:35 — Mate:627, Flush:317
356. 90327A125-M5x10mm-LowProfileSCS:36 — Mate:628, Mate:629, Flush:317
357. 90128A046-#2-.375in:7 — Mate:630, Flush:318, Mate:632, Mate:634
358. 90128A046-#2-.375in:8 — Mate:631, Flush:318, Mate:635
359. 90480A003-#2-HexNut:7 — Mate:635, Flush:319
360. 90480A003-#2-HexNut:8 — Mate:634, Flush:319, Angle:31, Mate:636
361. CNC-028-WireTrack1_MIR:1 — Mate:637, Mate:638, Mate:639, Mate:640, Mate:641, Mate:642, Mate:643
362. 91290A231-M5x15mm:131 — Mate:637, Flush:321
363. 91290A231-M5x15mm:132 — Mate:638, Flush:320, Flush:321
364. 91290A231-M5x15mm:133 — Mate:639, Mate:643, Flush:320
365. 10x15-CarbleCarrierXAxis-2924-1015-1000:1 [sub-assembly] — Mate:644, Angle:32, Mate:645, Mate:646, Mate:647, Mate:657, Mate:659, Mate:664
366. 94500A264-M3-12mm-ButtonHead:1 — Mate:646, Mate:647, Mate:652
367. 94500A264-M3-12mm-ButtonHead:2 — Mate:650, Mate:651, Mate:654
368. 94500A264-M3-12mm-ButtonHead:3 — Mate:648, Mate:649, Mate:655
369. 90576A102-M3-NylockNut:1 — Mate:652, Mate:653
370. 90576A102-M3-NylockNut:2 — Mate:655, Mate:656, Flush:322
371. 90576A102-M3-NylockNut:3 — Mate:654, Flush:322
372. CNC-030-XAxisCableCarrierMount:1 — Mate:657, Mate:658, Mate:659, Mate:660, Mate:661, Mate:662, Mate:663, Mate:666, Mate:668
373. 90327A125-M5x10mm-LowProfileSCS:37 — Mate:660, Mate:661
374. 94500A264-M3-12mm-ButtonHead:4 — Mate:662, Mate:664, Flush:323, Mate:665
375. 94500A264-M3-12mm-ButtonHead:5 — Mate:663, Flush:323, Mate:667
376. 90576A102-M3-NylockNut:4 — Mate:665, Mate:666, Flush:324
377. 90576A102-M3-NylockNut:5 — Mate:667, Flush:324
378. CNC-031-BackCover1:1 — Mate:671, Mate:672, Mate:673, Mate:674, Mate:675, Mate:690
379. 91290A198-M5-50mm:5 — Mate:673, Mate:674, Flush:326, Flush:328, Mate:678
380. 91290A198-M5-50mm:6 — Mate:675, Flush:326, Flush:333
381. CNC-031-BackCover1_MIR:1 — Mate:676, Mate:677, Mate:679, Mate:681
382. 91290A198-M5-50mm:7 — Mate:677, Flush:327, Mate:680
383. 91290A198-M5-50mm:8 — Mate:676, Flush:327, Flush:328
384. CNC-031-BackCover1_MIR2:1 — Mate:682, Mate:683, Mate:684, Mate:685, Mate:686, Mate:687, Mate:691
385. 91290A198-M5-50mm:9 — Mate:682, Flush:329
386. 91290A198-M5-50mm:10 — Mate:683, Mate:684, Flush:329, Flush:331
387. CNC-031-BackCover1_MIR_MIR3:1 — Mate:688, Mate:689
388. 91290A198-M5-50mm:11 — Mate:688, Flush:330, Flush:331
389. 91290A198-M5-50mm:12 — Mate:689, Flush:330
390. 91274A125-M5x8mm:49 — Mate:690, Flush:332, Flush:333
391. 91274A125-M5x8mm:50 — Mate:691, Flush:332
392. 91290A231-M5x15mm:20 — Mate:44, Mate:45
393. 91290A231-M5x15mm:21
394. 91290A231-M5x15mm:22 — Mate:264
395. 91290A231-M5x15mm:23 — Mate:302
396. 91290A231-M5x15mm:19 — Mate:42, Mate:43
397. 91290A231-M5x15mm:24
398. 91290A231-M5x15mm:25
399. 91290A231-M5x15mm:26
400. 91274A125-M5x8mm:1 — Mate:80, Mate:81
401. 91274A125-M5x8mm:2
402. 91274A125-M5x8mm:3
403. 91274A125-M5x8mm:4